# Autodesk Inventor assembly: curve+flat
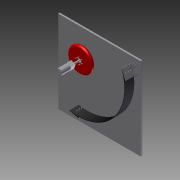
[picture p0: Inventor's stored thumbnail of the model, 180x180]
Saved by Autodesk Inventor 2011 SP1 (Build 150282100, 282)
## iProperties
Created: 2013-01-18
Part Number: curve+flat
Document SubType Name: Assembly
Designer: wes
Author: wes
## Documents named in this file (7)
- F:\ALL FILES\My Documents\GitHub\2013CAD\2013 robot\CurvedShooter\completed shooting platform.iam
- F:\ALL FILES\My Documents\GitHub\2013CAD\2013 robot\CurvedShooter\ajustableBase w mounting holes.ipt
- F:\ALL FILES\My Documents\GitHub\2013CAD\2013 robot\CurvedShooter\curveBracket.ipt
- F:\ALL FILES\My Documents\GitHub\2013CAD\2013 robot\CurvedShooter\Common Chassis Parts\.25 diameter 2'' bolt.ipt
- F:\ALL FILES\My Documents\GitHub\2013CAD\2013 robot\CurvedShooter\120 degree curved track.ipt
- F:\ALL FILES\My Documents\GitHub\2013CAD\2013 robot\CurvedShooter\Common Chassis Parts\.25 diameter 1'' bolt.ipt
- F:\ALL FILES\My Documents\GitHub\2013CAD\2013 robot\CurvedShooter\wheel+hub+axle.iam
## Components (19 placed, 6 different names)
1. ajustableBase w mounting holes:1 — Insert:14, Insert:15, Insert:16, Insert:17, Insert:18, Insert:19, Insert:24, Mate:2, Insert:33, Insert:34, Insert:35, Insert:36
2. curveBracket:1 — Insert:18, Insert:19, Mate:1, Insert:20, Insert:21, Insert:22, Insert:23
3. .25 diameter 2'' bolt:1 — Insert:14, Insert:33
4. .25 diameter 2'' bolt:2 — Insert:15, Insert:34
5. .25 diameter 2'' bolt:3 — Insert:17, Insert:36
6. .25 diameter 2'' bolt:4 — Insert:16, Insert:35
7. 120 degree curved track:1 — Mate:1, Insert:21, Insert:32
8. .25 diameter 1'' bolt:1 — Insert:23
9. .25 diameter 1'' bolt:2 — Insert:22
10. .25 diameter 1'' bolt:3 — Insert:20
11. wheel+hub+axle:1 [sub-assembly] — Insert:24
12. curveBracket:2 — Insert:25, Insert:26, Insert:27, Insert:28, Insert:29, Insert:30, Insert:31, Insert:32, Mate:2
13. .25 diameter 1'' bolt:4 — Insert:25
14. .25 diameter 1'' bolt:5 — Insert:26
15. .25 diameter 1'' bolt:6 — Insert:30
16. .25 diameter 1'' bolt:7 — Insert:31
17. .25 diameter 1'' bolt:8 — Insert:29
18. .25 diameter 1'' bolt:9 — Insert:28
19. .25 diameter 1'' bolt:10 — Insert:27
## Relationships (25: Insert 23, Mate 2)
- Insert:14: ajustableBase w mounting holes:1 ↔ .25 diameter 2'' bolt:1
- Insert:15: ajustableBase w mounting holes:1 ↔ .25 diameter 2'' bolt:2
- Insert:16: ajustableBase w mounting holes:1 ↔ .25 diameter 2'' bolt:4
- Insert:17: ajustableBase w mounting holes:1 ↔ .25 diameter 2'' bolt:3
- Insert:18: ajustableBase w mounting holes:1 ↔ curveBracket:1
- Insert:19: ajustableBase w mounting holes:1 ↔ curveBracket:1
- Mate:1: curveBracket:1 ↔ 120 degree curved track:1
- Insert:20: curveBracket:1 ↔ .25 diameter 1'' bolt:3
- Insert:21: curveBracket:1 ↔ 120 degree curved track:1
- Insert:22: curveBracket:1 ↔ .25 diameter 1'' bolt:2
- Insert:23: curveBracket:1 ↔ .25 diameter 1'' bolt:1
- Insert:24 (-76.2 mm): ajustableBase w mounting holes:1 ↔ wheel+hub+axle:1
- Insert:25: curveBracket:2 ↔ .25 diameter 1'' bolt:4
- Insert:26: curveBracket:2 ↔ .25 diameter 1'' bolt:5
- Insert:27: curveBracket:2 ↔ .25 diameter 1'' bolt:10
- Insert:28: curveBracket:2 ↔ .25 diameter 1'' bolt:9
- Insert:29: curveBracket:2 ↔ .25 diameter 1'' bolt:8
- Insert:30: curveBracket:2 ↔ .25 diameter 1'' bolt:6
- Insert:31: curveBracket:2 ↔ .25 diameter 1'' bolt:7
- Insert:32: 120 degree curved track:1 ↔ curveBracket:2
- Mate:2: ajustableBase w mounting holes:1 ↔ curveBracket:2
- Insert:33: ajustableBase w mounting holes:1 ↔ .25 diameter 2'' bolt:1
- Insert:34: ajustableBase w mounting holes:1 ↔ .25 diameter 2'' bolt:2
- Insert:35: ajustableBase w mounting holes:1 ↔ .25 diameter 2'' bolt:4
- Insert:36: ajustableBase w mounting holes:1 ↔ .25 diameter 2'' bolt:3
